# Autodesk Inventor assembly: lr_heater_assemble
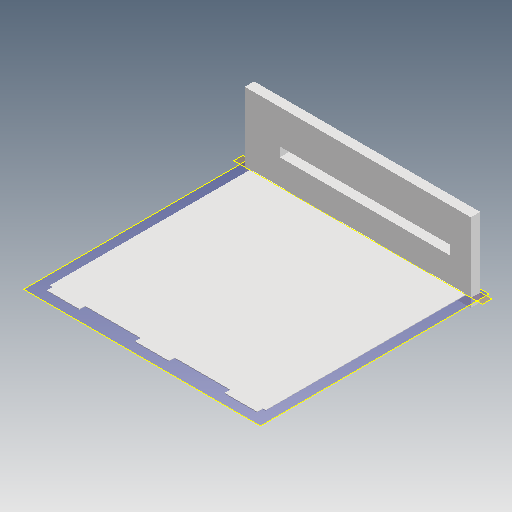
[picture p0: Inventor's stored thumbnail of the model, 512x512]
Saved by Autodesk Inventor 2020 (Build 240168000, 168)
## iProperties
Created: 2021-05-08
Part Number: lr_heater_assemble
Document SubType Name: Assembly
Designer: Hsu Daniel
Author: Hsu Daniel
## Documents named in this file (3)
- D:\Daniel\NTU\makeNTU2021\大改\lr_heater_assemble.iam
- D:\Daniel\NTU\makeNTU2021\大改\lr_heater.ipt
- D:\Daniel\NTU\makeNTU2021\大改\lr_bottom.ipt
## Components (2 placed, 2 different names)
1. lr_heater:1 — Mate:2, Mate:3, Mate:4
2. lr_bottom:1 — Mate:2, Mate:3, Mate:4
## Relationships (3: Mate 3)
- Mate:2: lr_heater:1 ↔ lr_bottom:1
- Mate:3: lr_heater:1 ↔ lr_bottom:1
- Mate:4: lr_heater:1 ↔ lr_bottom:1
